# Autodesk Inventor assembly: assembly.rev5
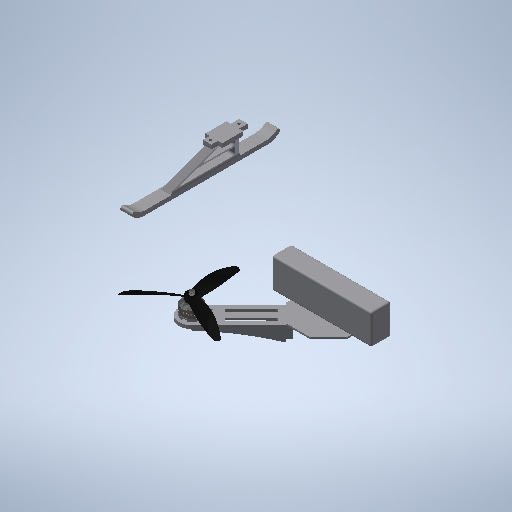
[picture p0: Inventor's stored thumbnail of the model, 512x512]
Saved by Autodesk Inventor 2025.2 (Build 292293000, 293)
## iProperties
Created: 2016-03-08
Part Number: assembly.rev5
Document SubType Name: Assembly
Designer: 200288284
Author: 200288284
## Documents named in this file (8)
- D:\UAV\esp drone\diy-drone\mechanical\完整体.iam
- D:\UAV\esp drone\diy-drone\mechanical\MOTOR_1806.iam
- D:\UAV\esp drone\diy-drone\mechanical\Tri-Blade 5045 Propeller\Tri-Blade 5045 Propeller\5045 CCW.ipt
- D:\UAV\esp drone\diy-drone\mechanical\电池.ipt
- D:\UAV\esp drone\diy-drone\mechanical\底板.ipt
- D:\UAV\esp drone\diy-drone\mechanical\新起落架.ipt
- D:\UAV\esp drone\diy-drone\mechanical\机臂.ipt
- D:\UAV\esp drone\diy-drone\mechanical\上板.ipt
## Components (7 placed, 7 different names)
1. 底板:1
2. 电池:2 — 配合:8, 表面齐平:1
3. MOTOR_1806:5 [sub-assembly] — 配合:3, 配合:4, 配合:5, 配合:6
4. 新起落架:1
5. 5045 CCW:8 — 配合:5, 配合:6
6. 机臂:1 — 配合:3, 配合:4, 配合:7, 配合:9, 表面齐平:2
7. 上板:1 — 配合:7, 配合:8, 表面齐平:1, 配合:9, 配合:10, 角度:1
## Relationships (11: Mate 8, Flush 2, Angle 1)
- 配合:3 [Mate]: MOTOR_1806:5 ↔ 机臂:1
- 配合:4 [Mate]: MOTOR_1806:5 ↔ 机臂:1
- 配合:5 [Mate]: MOTOR_1806:5 ↔ 5045 CCW:8
- 配合:6 [Mate]: MOTOR_1806:5 ↔ 5045 CCW:8
- 配合:7 [Mate]: 机臂:1 ↔ 上板:1
- 配合:8 [Mate]: 电池:2 ↔ 上板:1
- 表面齐平:1 [Flush] (23 mm): 电池:2 ↔ 上板:1
- 配合:9 [Mate]: 机臂:1 ↔ 上板:1
- 配合:10 [Mate]: 上板:1
- 角度:1 [Angle] (0 deg): 上板:1
- 表面齐平:2 [Flush]: 机臂:1
